# Autodesk Inventor assembly: FrisbeeShooter
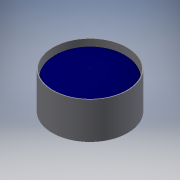
[picture p0: Inventor's stored thumbnail of the model, 180x180]
Saved by Autodesk Inventor 2016 (Build 200138000, 138)
## iProperties
Created: 2015-07-20
Part Number: FrisbeeShooter
Document SubType Name: Assembly
Designer: steele
Author: steele
## Documents named in this file (3)
- C:\snobotics\CAD-Development\robSteele\FRC 2013 Ultimate Ascent\FrisbeeShooter.iam
- C:\snobotics\CAD-Development\robSteele\FRC 2013 Ultimate Ascent\FrisbeeHopper.ipt
- C:\snobotics\ptc\FRC 2013 Ultimate Acsent\FRC_KOP\2013_frc_kop\Black Tote\53214-b_2013.ipt
## Components (2 placed, 2 different names)
1. FrisbeeHopper:1 — Insert:1
2. 53214-b_2013:1 — Insert:1
## Relationships (1: Insert 1)
- Insert:1: FrisbeeHopper:1 ↔ 53214-b_2013:1
